# Autodesk Inventor assembly: Assembly_Trial_3
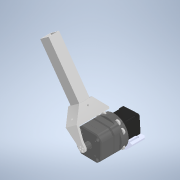
[picture p0: Inventor's stored thumbnail of the model, 180x180]
Saved by Autodesk Inventor 2022 (Build 260153000, 153)
## iProperties
Created: 2022-01-15
Part Number: Assembly_Trial_3
Document SubType Name: Assembly
Designer: Mlees
Author: Mlees
## Documents named in this file (18)
- C:\Users\Mlees\Desktop\504Engineering\Stepper-Servo_Based_Robotic_Arm\Assembly_Trial_3.iam
- C:\Users\Mlees\Desktop\504Engineering\Stepper-Servo_Based_Robotic_Arm\Downloaded Parts\nema17-speed-reducer-1.snapshot.9\24_Teeth_Sun_Gear.step.ipt
- C:\Users\Mlees\Desktop\504Engineering\Stepper-Servo_Based_Robotic_Arm\Downloaded Parts\nema17-speed-reducer-1.snapshot.9\36_Teeth_Planet_Gear.step.ipt
- C:\Users\Mlees\Desktop\504Engineering\Stepper-Servo_Based_Robotic_Arm\Downloaded Parts\nema17-speed-reducer-1.snapshot.9\96_Teeth_Gear.step.ipt
- C:\Users\Mlees\Desktop\504Engineering\Stepper-Servo_Based_Robotic_Arm\Downloaded Parts\nema17-speed-reducer-1.snapshot.9\Gear_Cover.ipt
- C:\Users\Mlees\Desktop\504Engineering\Stepper-Servo_Based_Robotic_Arm\Downloaded Parts\nema17-speed-reducer-1.snapshot.9\Plamet_Carrier.ipt
- C:\Users\Mlees\Desktop\504Engineering\Stepper-Servo_Based_Robotic_Arm\Downloaded Parts\90751A113_18-8 Stainless Steel Socket Head Screws.ipt
- C:\Users\Mlees\Desktop\504Engineering\Stepper-Servo_Based_Robotic_Arm\Downloaded Parts\nema-17-motor-mount-1.snapshot.1\NEMA_17_Bracket.ipt
- C:\Users\Mlees\Desktop\504Engineering\Stepper-Servo_Based_Robotic_Arm\Downloaded Parts\nema17-speed-reducer-1.snapshot.9\Thread Insert M3 x 6mm v2.step.iam
- C:\Users\Mlees\Desktop\504Engineering\Stepper-Servo_Based_Robotic_Arm\Downloaded Parts\Harmonic_Drive\Nema 17.ipt
- C:\Users\Mlees\Desktop\504Engineering\Stepper-Servo_Based_Robotic_Arm\Downloaded Parts\nema17-speed-reducer-1.snapshot.9\Gear_Cover_modified.ipt
- C:\Users\Mlees\Desktop\504Engineering\Stepper-Servo_Based_Robotic_Arm\Downloaded Parts\nema17-speed-reducer-1.snapshot.9\Plamet_Carrier_modified.ipt
- C:\Users\Mlees\Desktop\504Engineering\Stepper-Servo_Based_Robotic_Arm\Created Parts\OutPut_Shaft_From_Gearbox.ipt
- C:\Users\Mlees\Desktop\504Engineering\Stepper-Servo_Based_Robotic_Arm\Created Parts\604-2R2_Bearing4668K221_Permanently Lubricated Stainless Steel Ball Bearing.ipt
- C:\Users\Mlees\Desktop\504Engineering\Stepper-Servo_Based_Robotic_Arm\Downloaded Parts\nema17-speed-reducer-1.snapshot.9\96_Teeth_Gear.step_modified_bearings.ipt
- C:\Users\Mlees\Desktop\504Engineering\Stepper-Servo_Based_Robotic_Arm\Downloaded Parts\90666A106_Super-Corrosion-Resistant 316 Stainless Steel Socket Head Screw.ipt
- C:\Users\Mlees\Desktop\504Engineering\Stepper-Servo_Based_Robotic_Arm\Downloaded Parts\92855A844_18-8 Stainless Steel Low-Profile Socket Head Screws.ipt
- C:\Users\Mlees\Desktop\504Engineering\Stepper-Servo_Based_Robotic_Arm\Created Parts\Metal_Bone.ipt
## Components (50 placed, 17 different names)
1. 24_Teeth_Sun_Gear.step:1 — Rotational:11, Rotational:40
2. 36_Teeth_Planet_Gear.step:1 — Rotational:38
3. Gear_Cover:1 — Rigid:17, Rigid:18
4. Plamet_Carrier:1 — Rotational:37, Rotational:38, Rotational:39, Rotational:40, Rotational:41
5. 90751A113_18-8 Stainless Steel Socket Head Screws:3 — Rotational:50
6. NEMA_17_Bracket:1 — Rigid:12, Rotational:20
7. 36_Teeth_Planet_Gear.step:2 — Rotational:39
8. 36_Teeth_Planet_Gear.step:4 — Rotational:37
9. Thread Insert M3 x 6mm v2.step:1 [sub-assembly] — Rigid:16
10. Thread Insert M3 x 6mm v2.step:2 [sub-assembly] — Rigid:15
11. Thread Insert M3 x 6mm v2.step:3 [sub-assembly] — Rigid:13
12. Thread Insert M3 x 6mm v2.step:4 [sub-assembly] — Rotational:55
13. 90751A113_18-8 Stainless Steel Socket Head Screws:4 — Rotational:42
14. 90751A113_18-8 Stainless Steel Socket Head Screws:5 — Rotational:52
15. 90751A113_18-8 Stainless Steel Socket Head Screws:6 — Rotational:53
16. 90751A113_18-8 Stainless Steel Socket Head Screws:7 — Rotational:44
17. Nema 17:1 — Rigid:12, Rotational:11
18. 96_Teeth_Gear.step:2 — Rotational:16, Rotational:17, Rotational:18, Rotational:19, Rigid:18, Rotational:42, Rotational:43, Rotational:44, Rotational:45, Rigid:19
19. Thread Insert M3 x 6mm v2.step:5 [sub-assembly] — Rotational:16
20. Thread Insert M3 x 6mm v2.step:6 [sub-assembly] — Rotational:18
21. Thread Insert M3 x 6mm v2.step:7 [sub-assembly] — Rotational:19
22. Thread Insert M3 x 6mm v2.step:8 [sub-assembly] — Rotational:17
23. 24_Teeth_Sun_Gear.step:2 — Rotational:41, Rotational:49
24. 36_Teeth_Planet_Gear.step:5 — Rotational:46
25. 36_Teeth_Planet_Gear.step:6 — Rotational:48
26. 36_Teeth_Planet_Gear.step:7 — Rotational:47
27. 90751A113_18-8 Stainless Steel Socket Head Screws:12 — Rotational:51
28. 90751A113_18-8 Stainless Steel Socket Head Screws:14 — Rotational:45
29. 90751A113_18-8 Stainless Steel Socket Head Screws:15 — Rotational:43
30. Gear_Cover_modified:1 — Rigid:19, Rotational:50, Rotational:51, Rotational:52, Rotational:53
31. Plamet_Carrier_modified:1 — Rotational:46, Rotational:47, Rotational:48, Rotational:49, Rotational:54
32. OutPut_Shaft_From_Gearbox:1 — Rotational:54, Rigid:20
33. 604-2R2_Bearing4668K221_Permanently Lubricated Stainless Steel Ball Bearing:1 — Rotational:24
34. 604-2R2_Bearing4668K221_Permanently Lubricated Stainless Steel Ball Bearing:2 — Rotational:23
35. 604-2R2_Bearing4668K221_Permanently Lubricated Stainless Steel Ball Bearing:3 — Rotational:22
36. 96_Teeth_Gear.step_modified_bearings:1 — Rotational:20, Rotational:21, Rotational:22, Rotational:23, Rotational:24, Rotational:25, Rotational:26, Rotational:27, Rotational:28, Rotational:29, Rotational:30, Rotational:31, Rotational:32, Rotational:33, Rotational:34, Rotational:35, Rotational:36, Rigid:13, Rigid:15, Rigid:16, Rigid:17, Rotational:55
37. 604-2R2_Bearing4668K221_Permanently Lubricated Stainless Steel Ball Bearing:4 — Rotational:25
38. 604-2R2_Bearing4668K221_Permanently Lubricated Stainless Steel Ball Bearing:5 — Rotational:21
39. 604-2R2_Bearing4668K221_Permanently Lubricated Stainless Steel Ball Bearing:6 — Rotational:26
40. 90666A106_Super-Corrosion-Resistant 316 Stainless Steel Socket Head Screw:1 — Rotational:27
41. 90666A106_Super-Corrosion-Resistant 316 Stainless Steel Socket Head Screw:2 — Rotational:31
42. 90666A106_Super-Corrosion-Resistant 316 Stainless Steel Socket Head Screw:3 — Rotational:32
43. 90666A106_Super-Corrosion-Resistant 316 Stainless Steel Socket Head Screw:4 — Rotational:30
44. 90666A106_Super-Corrosion-Resistant 316 Stainless Steel Socket Head Screw:5 — Rotational:29
45. 90666A106_Super-Corrosion-Resistant 316 Stainless Steel Socket Head Screw:6 — Rotational:28
46. 92855A844_18-8 Stainless Steel Low-Profile Socket Head Screws:1 — Rotational:33
47. 92855A844_18-8 Stainless Steel Low-Profile Socket Head Screws:2 — Rotational:34
48. 92855A844_18-8 Stainless Steel Low-Profile Socket Head Screws:3 — Rotational:35
49. 92855A844_18-8 Stainless Steel Low-Profile Socket Head Screws:4 — Rotational:36
50. Metal_Bone:1 — Rigid:20
## Relationships (49: RevoluteJoint 41, WeldJoint 8)
- Rigid:12 [WeldJoint]: NEMA_17_Bracket:1 ↔ Nema 17:1
- Rotational:11 [RevoluteJoint]: 24_Teeth_Sun_Gear.step:1 ↔ Nema 17:1
- Rotational:16 [RevoluteJoint]: 96_Teeth_Gear.step:2 ↔ Thread Insert M3 x 6mm v2.step:5
- Rotational:17 [RevoluteJoint]: 96_Teeth_Gear.step:2 ↔ Thread Insert M3 x 6mm v2.step:8
- Rotational:18 [RevoluteJoint]: 96_Teeth_Gear.step:2 ↔ Thread Insert M3 x 6mm v2.step:6
- Rotational:19 [RevoluteJoint]: 96_Teeth_Gear.step:2 ↔ Thread Insert M3 x 6mm v2.step:7
- Rotational:20 [RevoluteJoint]: NEMA_17_Bracket:1 ↔ 96_Teeth_Gear.step_modified_bearings:1
- Rotational:21 [RevoluteJoint] (-0.25 mm): 96_Teeth_Gear.step_modified_bearings:1 ↔ 604-2R2_Bearing4668K221_Permanently Lubricated Stainless Steel Ball Bearing:5
- Rotational:22 [RevoluteJoint] (-0.25 mm): 604-2R2_Bearing4668K221_Permanently Lubricated Stainless Steel Ball Bearing:3 ↔ 96_Teeth_Gear.step_modified_bearings:1
- Rotational:23 [RevoluteJoint] (-0.25 mm): 604-2R2_Bearing4668K221_Permanently Lubricated Stainless Steel Ball Bearing:2 ↔ 96_Teeth_Gear.step_modified_bearings:1
- Rotational:24 [RevoluteJoint] (-0.25 mm): 604-2R2_Bearing4668K221_Permanently Lubricated Stainless Steel Ball Bearing:1 ↔ 96_Teeth_Gear.step_modified_bearings:1
- Rotational:25 [RevoluteJoint] (-0.25 mm): 96_Teeth_Gear.step_modified_bearings:1 ↔ 604-2R2_Bearing4668K221_Permanently Lubricated Stainless Steel Ball Bearing:4
- Rotational:26 [RevoluteJoint] (-0.25 mm): 96_Teeth_Gear.step_modified_bearings:1 ↔ 604-2R2_Bearing4668K221_Permanently Lubricated Stainless Steel Ball Bearing:6
- Rotational:27 [RevoluteJoint]: 96_Teeth_Gear.step_modified_bearings:1 ↔ 90666A106_Super-Corrosion-Resistant 316 Stainless Steel Socket Head Screw:1
- Rotational:28 [RevoluteJoint]: 96_Teeth_Gear.step_modified_bearings:1 ↔ 90666A106_Super-Corrosion-Resistant 316 Stainless Steel Socket Head Screw:6
- Rotational:29 [RevoluteJoint]: 96_Teeth_Gear.step_modified_bearings:1 ↔ 90666A106_Super-Corrosion-Resistant 316 Stainless Steel Socket Head Screw:5
- Rotational:30 [RevoluteJoint]: 96_Teeth_Gear.step_modified_bearings:1 ↔ 90666A106_Super-Corrosion-Resistant 316 Stainless Steel Socket Head Screw:4
- Rotational:31 [RevoluteJoint]: 96_Teeth_Gear.step_modified_bearings:1 ↔ 90666A106_Super-Corrosion-Resistant 316 Stainless Steel Socket Head Screw:2
- Rotational:32 [RevoluteJoint]: 96_Teeth_Gear.step_modified_bearings:1 ↔ 90666A106_Super-Corrosion-Resistant 316 Stainless Steel Socket Head Screw:3
- Rotational:33 [RevoluteJoint]: 96_Teeth_Gear.step_modified_bearings:1 ↔ 92855A844_18-8 Stainless Steel Low-Profile Socket Head Screws:1
- Rotational:34 [RevoluteJoint]: 96_Teeth_Gear.step_modified_bearings:1 ↔ 92855A844_18-8 Stainless Steel Low-Profile Socket Head Screws:2
- Rotational:35 [RevoluteJoint]: 96_Teeth_Gear.step_modified_bearings:1 ↔ 92855A844_18-8 Stainless Steel Low-Profile Socket Head Screws:3
- Rotational:36 [RevoluteJoint]: 96_Teeth_Gear.step_modified_bearings:1 ↔ 92855A844_18-8 Stainless Steel Low-Profile Socket Head Screws:4
- Rigid:13 [WeldJoint]: Thread Insert M3 x 6mm v2.step:3 ↔ 96_Teeth_Gear.step_modified_bearings:1
- Rigid:15 [WeldJoint]: Thread Insert M3 x 6mm v2.step:2 ↔ 96_Teeth_Gear.step_modified_bearings:1
- Rigid:16 [WeldJoint]: Thread Insert M3 x 6mm v2.step:1 ↔ 96_Teeth_Gear.step_modified_bearings:1
- Rotational:37 [RevoluteJoint]: Plamet_Carrier:1 ↔ 36_Teeth_Planet_Gear.step:4
- Rotational:38 [RevoluteJoint]: 36_Teeth_Planet_Gear.step:1 ↔ Plamet_Carrier:1
- Rotational:39 [RevoluteJoint]: Plamet_Carrier:1 ↔ 36_Teeth_Planet_Gear.step:2
- Rotational:40 [RevoluteJoint]: 24_Teeth_Sun_Gear.step:1 ↔ Plamet_Carrier:1
- Rigid:17 [WeldJoint]: Gear_Cover:1 ↔ 96_Teeth_Gear.step_modified_bearings:1
- Rigid:18 [WeldJoint]: Gear_Cover:1 ↔ 96_Teeth_Gear.step:2
- Rotational:41 [RevoluteJoint]: Plamet_Carrier:1 ↔ 24_Teeth_Sun_Gear.step:2
- Rotational:42 [RevoluteJoint]: 90751A113_18-8 Stainless Steel Socket Head Screws:4 ↔ 96_Teeth_Gear.step:2
- Rotational:43 [RevoluteJoint]: 96_Teeth_Gear.step:2 ↔ 90751A113_18-8 Stainless Steel Socket Head Screws:15
- Rotational:44 [RevoluteJoint]: 90751A113_18-8 Stainless Steel Socket Head Screws:7 ↔ 96_Teeth_Gear.step:2
- Rotational:45 [RevoluteJoint]: 96_Teeth_Gear.step:2 ↔ 90751A113_18-8 Stainless Steel Socket Head Screws:14
- Rotational:46 [RevoluteJoint]: 36_Teeth_Planet_Gear.step:5 ↔ Plamet_Carrier_modified:1
- Rotational:47 [RevoluteJoint]: 36_Teeth_Planet_Gear.step:7 ↔ Plamet_Carrier_modified:1
- Rotational:48 [RevoluteJoint]: 36_Teeth_Planet_Gear.step:6 ↔ Plamet_Carrier_modified:1
- Rotational:49 [RevoluteJoint]: 24_Teeth_Sun_Gear.step:2 ↔ Plamet_Carrier_modified:1
- Rigid:19 [WeldJoint]: 96_Teeth_Gear.step:2 ↔ Gear_Cover_modified:1
- Rotational:50 [RevoluteJoint]: 90751A113_18-8 Stainless Steel Socket Head Screws:3 ↔ Gear_Cover_modified:1
- Rotational:51 [RevoluteJoint]: 90751A113_18-8 Stainless Steel Socket Head Screws:12 ↔ Gear_Cover_modified:1
- Rotational:52 [RevoluteJoint]: 90751A113_18-8 Stainless Steel Socket Head Screws:5 ↔ Gear_Cover_modified:1
- Rotational:53 [RevoluteJoint]: 90751A113_18-8 Stainless Steel Socket Head Screws:6 ↔ Gear_Cover_modified:1
- Rotational:54 [RevoluteJoint]: Plamet_Carrier_modified:1 ↔ OutPut_Shaft_From_Gearbox:1
- Rotational:55 [RevoluteJoint]: Thread Insert M3 x 6mm v2.step:4 ↔ 96_Teeth_Gear.step_modified_bearings:1
- Rigid:20 [WeldJoint]: OutPut_Shaft_From_Gearbox:1 ↔ Metal_Bone:1
